# Autodesk Inventor assembly: Dilution Printer
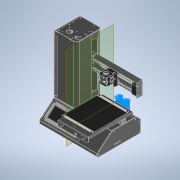
[picture p0: Inventor's stored thumbnail of the model, 180x180]
Saved by Autodesk Inventor 2022 (Build 260153000, 153)
## iProperties
Created: 2021-12-01
Part Number: Dilution Printer
Document SubType Name: Assembly
Designer: efred
Author: efred
## Documents named in this file (8)
- C:\Users\efred\OneDrive - Imperial College London\ROBOICP\Final Assembly\Dilution Printer.iam
- C:\Users\efred\OneDrive - Imperial College London\ROBOICP\Final Assembly\Base_v7.ipt
- C:\Users\efred\OneDrive - Imperial College London\ROBOICP\Final Assembly\Bed_Base_v2.ipt
- C:\Users\efred\OneDrive - Imperial College London\ROBOICP\Final Assembly\Bed_Surface_v3.ipt
- C:\Users\efred\OneDrive - Imperial College London\ROBOICP\Final Assembly\Control_Panel_v4.ipt
- C:\Users\efred\OneDrive - Imperial College London\ROBOICP\Final Assembly\Print_Head_v5.ipt
- C:\Users\efred\OneDrive - Imperial College London\ROBOICP\Final Assembly\Tower_v7.ipt
- C:\Users\efred\OneDrive - Imperial College London\ROBOICP\Final Assembly\X_Axis_v8.ipt
## Components (7 placed, 7 different names)
1. Base_v7:1 — Mate:1, Mate:2, Angle:1, Mate:3, Mate:4, Mate:5, Flush:1, Mate:6, Mate:7, Symmetry:1
2. Bed_Base_v2:1 — Mate:3, Mate:4, Mate:5, Mate:8, Mate:9, Mate:10
3. Bed_Surface_v3:1 — Mate:8, Mate:9, Mate:10
4. Control_Panel_v4:1 — Mate:1, Mate:2, Angle:1
5. Print_Head_v5:1 — Mate:13, Mate:14, Mate:15
6. Tower_v7:1 — Flush:1, Mate:6, Mate:7, Mate:11, Mate:12, Symmetry:1, Mate:16
7. X_Axis_v8:1 — Mate:11, Mate:12, Mate:13, Mate:14, Mate:15, Mate:16
## Relationships (19: Mate 16, Angle 1, Flush 1, Symmetry 1)
- Mate:1: Base_v7:1 ↔ Control_Panel_v4:1
- Mate:2: Base_v7:1 ↔ Control_Panel_v4:1
- Angle:1 (180 deg): Base_v7:1 ↔ Control_Panel_v4:1
- Mate:3: Base_v7:1 ↔ Bed_Base_v2:1
- Mate:4: Base_v7:1 ↔ Bed_Base_v2:1
- Mate:5: Base_v7:1 ↔ Bed_Base_v2:1
- Flush:1: Base_v7:1 ↔ Tower_v7:1
- Mate:6: Base_v7:1 ↔ Tower_v7:1
- Mate:7: Base_v7:1 ↔ Tower_v7:1
- Mate:8: Bed_Base_v2:1 ↔ Bed_Surface_v3:1
- Mate:9: Bed_Base_v2:1 ↔ Bed_Surface_v3:1
- Mate:10: Bed_Base_v2:1 ↔ Bed_Surface_v3:1
- Mate:11: Tower_v7:1 ↔ X_Axis_v8:1
- Mate:12: Tower_v7:1 ↔ X_Axis_v8:1
- Mate:13: Print_Head_v5:1 ↔ X_Axis_v8:1
- Mate:14: Print_Head_v5:1 ↔ X_Axis_v8:1
- Symmetry:1: Base_v7:1 ↔ Tower_v7:1
- Mate:15: Print_Head_v5:1 ↔ X_Axis_v8:1
- Mate:16: Tower_v7:1 ↔ X_Axis_v8:1
